# Autodesk Inventor assembly: mid_assem
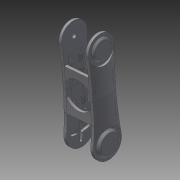
[picture p0: Inventor's stored thumbnail of the model, 180x180]
Saved by Autodesk Inventor 2014 (Build 180170000, 170)
## iProperties
Created: 2014-04-24
Part Number: mid_assem
Document SubType Name: Assembly
Designer: t_emanb
Author: t_emanb
## Documents named in this file (7)
- C:\Users\t_emanb\Documents\3D printed arm\4th version\mid_assem.iam
- C:\Users\t_emanb\Documents\3D printed arm\4th version\mid_curveLhorn.ipt
- C:\Users\t_emanb\Documents\3D printed arm\4th version\mid_curveLpin.ipt
- C:\Users\t_emanb\Documents\3D printed arm\4th version\mid_curveUhorn.ipt
- C:\Users\t_emanb\Documents\3D printed arm\4th version\mid_curveUpin.ipt
- C:\Users\t_emanb\Documents\3D printed arm\4th version\mid_braceL.ipt
- C:\Users\t_emanb\Documents\3D printed arm\4th version\mid_braceU.ipt
## Components (8 placed, 6 different names)
1. mid_curveLhorn:1 — Flush:1, Mate:1, Mate:2, Mate:5, Mate:10, Mate:11, Mate:13
2. mid_curveLpin:1 — Flush:2, Mate:3, Mate:4, Mate:8, Mate:9, Angle:1, Mate:22
3. mid_curveUhorn:1 — Flush:2, Mate:3, Mate:4, Mate:16, Mate:19
4. mid_curveUpin:1 — Flush:1, Mate:1, Mate:2, Mate:14, Mate:17, Angle:1, Mate:20, Mate:21
5. mid_braceL:1 — Mate:5, Mate:8, Mate:9, Mate:10
6. mid_braceL:2 — Mate:11, Mate:13, Mate:22
7. mid_braceU:1 — Mate:14, Mate:16, Mate:21
8. mid_braceU:2 — Mate:17, Mate:19, Mate:20
## Relationships (20: Mate 17, Flush 2, Angle 1)
- Flush:1: mid_curveLhorn:1 ↔ mid_curveUpin:1
- Mate:1: mid_curveLhorn:1 ↔ mid_curveUpin:1
- Mate:2: mid_curveLhorn:1 ↔ mid_curveUpin:1
- Flush:2: mid_curveLpin:1 ↔ mid_curveUhorn:1
- Mate:3: mid_curveLpin:1 ↔ mid_curveUhorn:1
- Mate:4: mid_curveLpin:1 ↔ mid_curveUhorn:1
- Mate:5: mid_curveLhorn:1 ↔ mid_braceL:1
- Mate:8: mid_curveLpin:1 ↔ mid_braceL:1
- Mate:9: mid_curveLpin:1 ↔ mid_braceL:1
- Mate:10: mid_curveLhorn:1 ↔ mid_braceL:1
- Mate:11: mid_curveLhorn:1 ↔ mid_braceL:2
- Mate:13: mid_curveLhorn:1 ↔ mid_braceL:2
- Mate:14: mid_curveUpin:1 ↔ mid_braceU:1
- Mate:16: mid_curveUhorn:1 ↔ mid_braceU:1
- Mate:17: mid_curveUpin:1 ↔ mid_braceU:2
- Mate:19: mid_curveUhorn:1 ↔ mid_braceU:2
- Angle:1 (180 deg): mid_curveLpin:1 ↔ mid_curveUpin:1
- Mate:20: mid_curveUpin:1 ↔ mid_braceU:2
- Mate:21: mid_curveUpin:1 ↔ mid_braceU:1
- Mate:22: mid_curveLpin:1 ↔ mid_braceL:2
